# Autodesk Inventor assembly: RAW gearbox
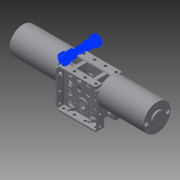
[picture p0: Inventor's stored thumbnail of the model, 180x180]
Saved by Autodesk Inventor 2015 SP1 (Build 190203100, 203)
## iProperties
Created: 2015-01-17
Part Number: RAW gearbox
Document SubType Name: Assembly
Designer: Admin
Title: 14 to 1 worm gearbox AB.STEP
Description: STEP AP203
Creation Date: 2013-08-05
Sending System: SolidWorks 2010
Preprocessor: SwSTEP 2.0
Author: Admin
## Documents named in this file (15)
- C:\Users\Admin\Desktop\Jarod's LEXAR Backup\Robotics\FRC\2015\CAD\Robot\Chassis\Imported Components\RAW gearbox\RAW gearbox.iam
- C:\Users\Admin\Desktop\Jarod's LEXAR Backup\Robotics\FRC\2015\CAD\Robot\Chassis\Imported Components\RAW gearbox\10-32x1750_shcs_HX-SHCS 0.19-32x1.375x1-C.ipt
- C:\Users\Admin\Desktop\Jarod's LEXAR Backup\Robotics\FRC\2015\CAD\Robot\Chassis\Imported Components\RAW gearbox\8mm_spring_clip am-0033.ipt
- C:\Users\Admin\Desktop\Jarod's LEXAR Backup\Robotics\FRC\2015\CAD\Robot\Chassis\Imported Components\RAW gearbox\5-16 washer_smart.ipt
- C:\Users\Admin\Desktop\Jarod's LEXAR Backup\Robotics\FRC\2015\CAD\Robot\Chassis\Imported Components\RAW gearbox\2mm x 2mm x 10mm Machine Key_smart.ipt
- C:\Users\Admin\Desktop\Jarod's LEXAR Backup\Robotics\FRC\2015\CAD\Robot\Chassis\Imported Components\RAW gearbox\Spacer Plate AB.ipt
- C:\Users\Admin\Desktop\Jarod's LEXAR Backup\Robotics\FRC\2015\CAD\Robot\Chassis\Imported Components\RAW gearbox\RAW worm shaft.iam
- C:\Users\Admin\Desktop\Jarod's LEXAR Backup\Robotics\FRC\2015\CAD\Robot\Chassis\Imported Components\RAW gearbox\Spur gear 20DP 12T 14.5PA .515FW_Spur gear 20DP 12T 14.5PA .515FW.ipt
- C:\Users\Admin\Desktop\Jarod's LEXAR Backup\Robotics\FRC\2015\CAD\Robot\Chassis\Imported Components\RAW gearbox\SHCS 10-32 x 0.625.ipt
- C:\Users\Admin\Desktop\Jarod's LEXAR Backup\Robotics\FRC\2015\CAD\Robot\Chassis\Imported Components\RAW gearbox\CIM motor-1.ipt
- C:\Users\Admin\Desktop\Jarod's LEXAR Backup\Robotics\FRC\2015\CAD\Robot\Chassis\Imported Components\RAW gearbox\10-32 Nylock Nut 1_90631A411.ipt
- C:\Users\Admin\Desktop\Jarod's LEXAR Backup\Robotics\FRC\2015\CAD\Robot\Chassis\Imported Components\RAW gearbox\outside plate AB.ipt
- C:\Users\Admin\Desktop\Jarod's LEXAR Backup\Robotics\FRC\2015\CAD\Robot\Chassis\Imported Components\RAW gearbox\WormGearSpacer-1.ipt
- C:\Users\Admin\Desktop\Jarod's LEXAR Backup\Robotics\FRC\2015\CAD\Robot\Chassis\Imported Components\RAW gearbox\WormGear-1.ipt
- C:\Users\Admin\Desktop\Jarod's LEXAR Backup\Robotics\FRC\2015\CAD\Robot\Chassis\Imported Components\RAW gearbox\-5 hex bearing-1.ipt
## Components (32 placed, 32 different names)
1. 10-32x1750_shcs_HX-SHCS 0.19-32x1.375x1-C_1
2. 8mm_spring_clip am-0033_2
3. 5-16 washer_smart_4
4. 10-32x1750_shcs_HX-SHCS 0.19-32x1.375x1-C_5
5. 2mm x 2mm x 10mm Machine Key_smart_6
6. Spacer Plate AB_8 — Mate:1
7. 10-32x1750_shcs_HX-SHCS 0.19-32x1.375x1-C_9
8. 2mm x 2mm x 10mm Machine Key_smart_10
9. RAW worm shaft_11 [sub-assembly] — Mate:1, Mate:2
10. 10-32x1750_shcs_HX-SHCS 0.19-32x1.375x1-C_13
11. Spur gear 20DP 12T 14.5PA .515FW_Spur gear 20DP 12T 14.5PA .515FW_14
12. Spacer Plate AB_15 — Mate:2
13. SHCS 10-32 x 0.625_16
14. CIM motor-1_17
15. SHCS 10-32 x 0.625_18
16. 8mm_spring_clip am-0033_19
17. CIM motor-1_20
18. 10-32 Nylock Nut 1_90631A411_21
19. outside plate AB_22 — Mate:3, Mate:4
20. 10-32 Nylock Nut 1_90631A411_23
21. WormGearSpacer-1_24
22. SHCS 10-32 x 0.625_25
23. outside plate AB_26
24. 10-32 Nylock Nut 1_90631A411_27
25. WormGear-1_28
26. SHCS 10-32 x 0.625_29
27. WormGearSpacer-1_30
28. 10-32 Nylock Nut 1_90631A411_31
29. Spur gear 20DP 12T 14.5PA .515FW_Spur gear 20DP 12T 14.5PA .515FW_32
30. -5 hex bearing-1_33
31. 5-16 washer_smart_34
32. -5 hex bearing-1:2 — Mate:3, Mate:4
## Relationships (4: Mate 4)
- Mate:1: Spacer Plate AB_8 ↔ RAW worm shaft_11
- Mate:2: RAW worm shaft_11 ↔ Spacer Plate AB_15
- Mate:3: outside plate AB_22 ↔ -5 hex bearing-1:2
- Mate:4: outside plate AB_22 ↔ -5 hex bearing-1:2
